# Autodesk Inventor assembly: Felga2XForma
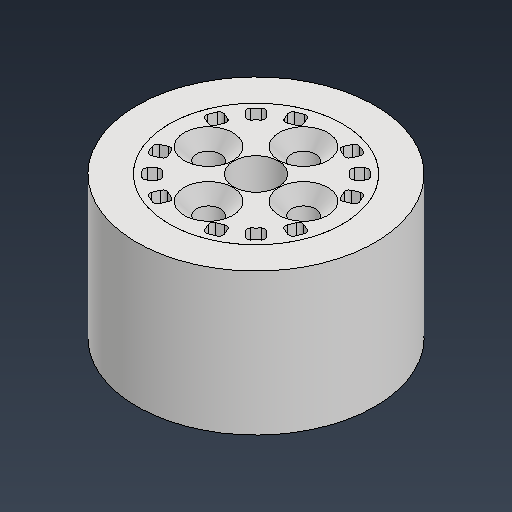
[picture p0: Inventor's stored thumbnail of the model, 512x512]
Saved by Autodesk Inventor 2026.2 (Build 302298010, 298A)
## iProperties
Created: 2026-08-04
Part Number: Felga2XForma
Document SubType Name: Assembly
Designer: szymo
Author: szymo
## Documents named in this file (3)
- D:\tech\robotyka\robots\evangelion-turbo\inventor-project\Felga2XForma.iam
- D:\tech\robotyka\robots\evangelion-turbo\inventor-project\Felga2.ipt
- D:\tech\robotyka\robots\evangelion-turbo\inventor-project\FelgaForma.ipt
## Components (2 placed, 2 different names)
1. Felga2:1 — Flush:1
2. FelgaForma:1 — Flush:1
## Relationships (1: Flush 1)
- Flush:1: Felga2:1 ↔ FelgaForma:1
